# Autodesk Inventor assembly: fight_robot_fin2
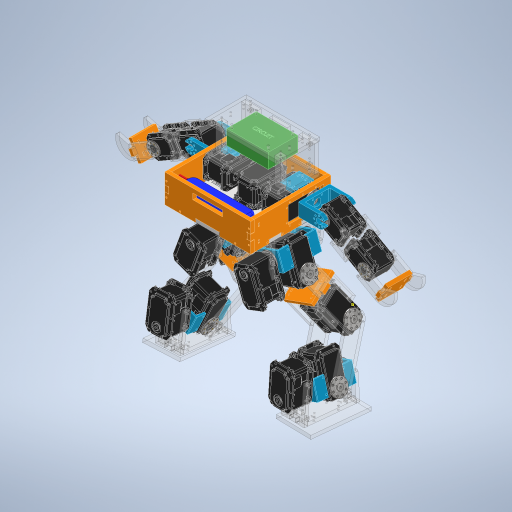
[picture p0: Inventor's stored thumbnail of the model, 512x512]
Saved by Autodesk Inventor 2024 (Build 280153000, 153)
## iProperties
Created: 2024-09-16
Part Number: fight_robot_fin2
Document SubType Name: Assembly
Designer: jmha0
Author: jmha0
## Documents named in this file (15)
- C:\Users\jmha0\OneDrive\바탕 화면\19th_intern_hjm_fight_robot\부품\fight_robot_fin2.iam
- C:\Users\jmha0\OneDrive\바탕 화면\19th_intern_hjm_fight_robot\부품\Lower_Body\waist\waist_fin1.iam
- C:\Users\jmha0\OneDrive\바탕 화면\19th_intern_hjm_fight_robot\부품\Lower_Body\pelvis_w_motor\pelvis_w_motor_fin1.iam
- C:\Users\jmha0\OneDrive\바탕 화면\19th_intern_hjm_fight_robot\부품\Lower_Body\pelvis_w_motor\pelvis_w_motor_fin1_opp.iam
- C:\Users\jmha0\OneDrive\바탕 화면\19th_intern_hjm_fight_robot\부품\Lower_Body\knee_w_motor\knee_fin1.iam
- C:\Users\jmha0\OneDrive\바탕 화면\19th_intern_hjm_fight_robot\부품\Lower_Body\ankle_w_feet\ankle_w_feet_right.iam
- C:\Users\jmha0\OneDrive\바탕 화면\19th_intern_hjm_fight_robot\부품\Lower_Body\ankle_w_feet\ankle_w_feet_left.iam
- C:\Users\jmha0\OneDrive\바탕 화면\19th_intern_hjm_fight_robot\부품\Upper_Body\etc\long_horn1.ipt
- C:\Users\jmha0\OneDrive\바탕 화면\19th_intern_hjm_fight_robot\부품\Upper_Body\arm\arm_fin_left1.iam
- C:\Users\jmha0\OneDrive\바탕 화면\19th_intern_hjm_fight_robot\부품\Upper_Body\arm\arm_fin_right1.iam
- C:\Users\jmha0\OneDrive\바탕 화면\19th_intern_hjm_fight_robot\부품\Upper_Body\hand\hand_fin1_opp.iam
- C:\Users\jmha0\OneDrive\바탕 화면\19th_intern_hjm_fight_robot\부품\Upper_Body\hand\hand_fin1.iam
- C:\Users\jmha0\OneDrive\바탕 화면\19th_intern_hjm_fight_robot\부품\battery\Enrichpower_2200mAh_11.1V_30C.ipt
- C:\Users\jmha0\OneDrive\바탕 화면\19th_intern_hjm_fight_robot\부품\circuit\Circuit.ipt
- C:\Users\jmha0\OneDrive\바탕 화면\19th_intern_hjm_fight_robot\부품\Upper_Body\Upper_w_head\upper_w_head_fin1.iam
## Components (15 placed, 14 different names)
1. waist_fin1:1 [sub-assembly] — 메이트:1, 각도:1, 메이트:2, 각도:2, 각도:3, 각도:4, 삽입:5, 삽입:6, 삽입:18
2. pelvis_w_motor_fin1:1 [sub-assembly] — 메이트:2, 각도:2, 각도:3, 삽입:1, 삽입:2
3. pelvis_w_motor_fin1_opp:1 [sub-assembly] — 메이트:1, 각도:1, 각도:4, 삽입:3, 삽입:4
4. knee_fin1:1 [sub-assembly] — 삽입:3, 삽입:4, 메이트:3, 메이트:4
5. knee_fin1:2 [sub-assembly] — 삽입:1, 삽입:2, 메이트:5, 메이트:6
6. ankle_w_feet_right:1 [sub-assembly] — 메이트:3, 메이트:4
7. ankle_w_feet_left:1 [sub-assembly] — 메이트:5, 메이트:6
8. long_horn1:1 — 삽입:5, 삽입:6, 삽입:17, 삽입:18
9. arm_fin_left1:1 [sub-assembly] — 삽입:13, 삽입:14, 삽입:19
10. arm_fin_right1:1 [sub-assembly] — 삽입:15, 삽입:16, 삽입:20
11. hand_fin1_opp:1 [sub-assembly] — 삽입:15, 삽입:16
12. hand_fin1:1 [sub-assembly] — 삽입:13, 삽입:14
13. Enrichpower_2200mAh_11.1V_30C:1
14. Circuit:1 — 삽입:21, 삽입:22
15. upper_w_head_fin1:1 [sub-assembly] — 삽입:17, 삽입:19, 삽입:20, 삽입:21, 삽입:22
## Relationships (26: Insert 16, Mate 6, Angle 4)
- 메이트:1 [Mate]: waist_fin1:1 ↔ pelvis_w_motor_fin1_opp:1
- 각도:1 [Angle] (0 deg): waist_fin1:1 ↔ pelvis_w_motor_fin1_opp:1
- 메이트:2 [Mate]: waist_fin1:1 ↔ pelvis_w_motor_fin1:1
- 각도:2 [Angle] (0 deg): waist_fin1:1 ↔ pelvis_w_motor_fin1:1
- 각도:3 [Angle] (-20 deg): waist_fin1:1 ↔ pelvis_w_motor_fin1:1
- 각도:4 [Angle] (20 deg): waist_fin1:1 ↔ pelvis_w_motor_fin1_opp:1
- 삽입:1 [Insert]: pelvis_w_motor_fin1:1 ↔ knee_fin1:2
- 삽입:2 [Insert]: pelvis_w_motor_fin1:1 ↔ knee_fin1:2
- 삽입:3 [Insert]: pelvis_w_motor_fin1_opp:1 ↔ knee_fin1:1
- 삽입:4 [Insert]: pelvis_w_motor_fin1_opp:1 ↔ knee_fin1:1
- 메이트:3 [Mate]: knee_fin1:1 ↔ ankle_w_feet_right:1
- 메이트:4 [Mate]: knee_fin1:1 ↔ ankle_w_feet_right:1
- 메이트:5 [Mate]: knee_fin1:2 ↔ ankle_w_feet_left:1
- 메이트:6 [Mate]: knee_fin1:2 ↔ ankle_w_feet_left:1
- 삽입:5 [Insert]: waist_fin1:1 ↔ long_horn1:1
- 삽입:6 [Insert]: waist_fin1:1 ↔ long_horn1:1
- 삽입:13 [Insert]: arm_fin_left1:1 ↔ hand_fin1:1
- 삽입:14 [Insert]: arm_fin_left1:1 ↔ hand_fin1:1
- 삽입:15 [Insert]: arm_fin_right1:1 ↔ hand_fin1_opp:1
- 삽입:16 [Insert]: arm_fin_right1:1 ↔ hand_fin1_opp:1
- 삽입:17 [Insert]: long_horn1:1 ↔ upper_w_head_fin1:1
- 삽입:18 [Insert]: waist_fin1:1 ↔ long_horn1:1
- 삽입:19 [Insert]: arm_fin_left1:1 ↔ upper_w_head_fin1:1
- 삽입:20 [Insert]: arm_fin_right1:1 ↔ upper_w_head_fin1:1
- 삽입:21 [Insert]: Circuit:1 ↔ upper_w_head_fin1:1
- 삽입:22 [Insert]: Circuit:1 ↔ upper_w_head_fin1:1
